# Autodesk Inventor assembly: Naroznik
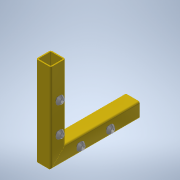
[picture p0: Inventor's stored thumbnail of the model, 180x180]
Saved by Autodesk Inventor 2021 (Build 250183000, 183)
## iProperties
Created: 2024-04-18
Part Number: Naroznik
Document SubType Name: Assembly
Designer: Michal
Author: Michal
## Documents named in this file (4)
- C:\Users\Michal\Documents\GitHub\PNW_PhotoBoothFrame_3D\Naroznik.iam
- C:\Users\Michal\Documents\GitHub\PNW_PhotoBoothFrame_3D\Naroznik profil 1.ipt
- C:\Users\Michal\Documents\GitHub\PNW_PhotoBoothFrame_3D\Naroznik profil 2.ipt
- C:\Users\Michal\Documents\GitHub\PNW_PhotoBoothFrame_3D\M8x15.ipt
## Components (6 placed, 3 different names)
1. Naroznik profil 2:1 — Mate:1, Flush:1, Mate:2, Mate:3, Mate:4, Mate:7
2. Naroznik profil 1:1 — Mate:1, Flush:1, Mate:2, Mate:5, Mate:6
3. M8x15:1 — Mate:3, Flush:2, Flush:3, Flush:4, Mate:7
4. M8x15:2 — Mate:4, Flush:2
5. M8x15:3 — Mate:5, Flush:3
6. M8x15:4 — Mate:6, Flush:4
## Relationships (11: Mate 7, Flush 4)
- Mate:1: Naroznik profil 2:1 ↔ Naroznik profil 1:1
- Flush:1: Naroznik profil 2:1 ↔ Naroznik profil 1:1
- Mate:2: Naroznik profil 2:1 ↔ Naroznik profil 1:1
- Mate:3: Naroznik profil 2:1 ↔ M8x15:1
- Mate:4: Naroznik profil 2:1 ↔ M8x15:2
- Mate:5: Naroznik profil 1:1 ↔ M8x15:3
- Mate:6: Naroznik profil 1:1 ↔ M8x15:4
- Flush:2: M8x15:1 ↔ M8x15:2
- Flush:3: M8x15:1 ↔ M8x15:3
- Flush:4: M8x15:1 ↔ M8x15:4
- Mate:7 (3 mm): Naroznik profil 2:1 ↔ M8x15:1
